# Autodesk Inventor assembly: ForearmActuatorConnector
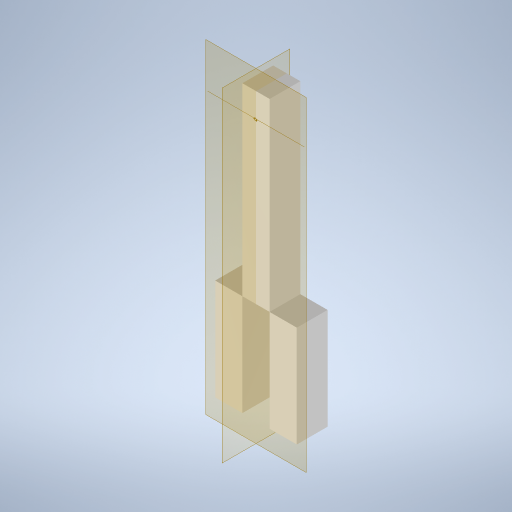
[picture p0: Inventor's stored thumbnail of the model, 512x512]
Saved by Autodesk Inventor 2023 (Build 270158000, 158)
## iProperties
Created: 2023-03-27
Part Number: ForearmActuatorConnector
Document SubType Name: Assembly
Designer: LattePanda
Author: LattePanda
## Documents named in this file (3)
- C:\Users\LattePanda\Desktop\str1ker\description\models\src\ForearmActuatorConnector.iam
- C:\Users\LattePanda\Desktop\str1ker\parts\ForearmActuatorConnector.ipt
- C:\Users\LattePanda\Desktop\str1ker\description\models\src\ForearmActuatorConnectorBoundingBox.ipt
## Components (3 placed, 2 different names)
1. ForearmActuatorConnector:1 — Mate:1, Mate:2, Mate:3
2. ForearmActuatorConnector:2 — Flush:1, Mate:2
3. ForearmActuatorConnectorBoundingBox:1 — Flush:2
## Relationships (5: Mate 3, Flush 2)
- Flush:1 (0.64 mm): ForearmActuatorConnector:2
- Mate:1 (0.64 mm): ForearmActuatorConnector:1
- Mate:2: ForearmActuatorConnector:1 ↔ ForearmActuatorConnector:2
- Mate:3: ForearmActuatorConnector:1
- Flush:2: ForearmActuatorConnectorBoundingBox:1
